# Autodesk Inventor assembly: gurav2 assembly
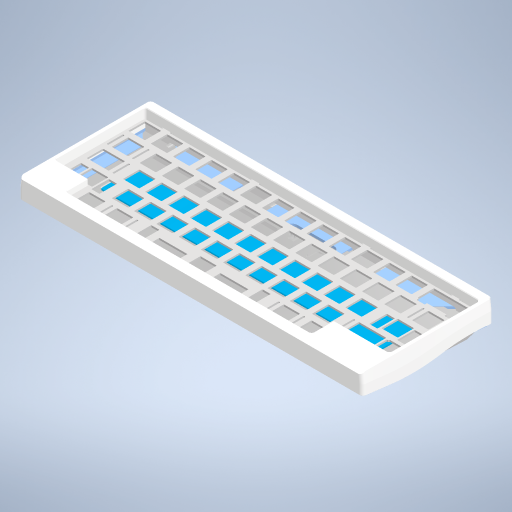
[picture p0: Inventor's stored thumbnail of the model, 512x512]
Saved by Autodesk Inventor 2023 (Build 270158000, 158)
## iProperties
Created: 2023-10-18
Part Number: gurav2 assembly
Document SubType Name: Assembly
Designer: Eric
Author: Eric
## Documents named in this file (8)
- C:\Users\Eric\Desktop\guracase\v2 Parts\gurav2 assembly.iam
- C:\Users\Eric\Desktop\guracase\v2 Parts\bottomcase.ipt
- C:\Users\Eric\Desktop\guracase\v2 Parts\rightdiffuser.ipt
- C:\Users\Eric\Desktop\guracase\v2 Parts\leftdiffuser.ipt
- C:\Users\Eric\Desktop\guracase\v2 Parts\reardiffuser.ipt
- C:\Users\Eric\Desktop\guracase\v2 Parts\weight.ipt
- C:\Users\Eric\Desktop\guracase\v2 Parts\topcase.ipt
- C:\Users\Eric\Desktop\guracase\v2 Parts\hhkbplate.ipt
## Components (7 placed, 7 different names)
1. bottomcase:1 — Mate:1, Mate:2, Mate:3, Mate:4, Mate:5, Mate:6, Mate:7, Mate:8, Flush:1, Mate:9, Mate:10, Flush:2, Mate:11, Mate:13
2. rightdiffuser:1 — Mate:1, Mate:2, Mate:3, Mate:12
3. leftdiffuser:1 — Mate:4, Mate:5, Mate:6
4. reardiffuser:1 — Mate:7, Mate:8, Flush:1
5. weight:1 — Mate:9, Mate:10, Flush:2
6. topcase:1 — Mate:11, Mate:12, Mate:13, Mate:14, Mate:15
7. hhkbplate:1 — Mate:14, Mate:15
## Relationships (17: Mate 15, Flush 2)
- Mate:1: bottomcase:1 ↔ rightdiffuser:1
- Mate:2 (0.125 mm): bottomcase:1 ↔ rightdiffuser:1
- Mate:3 (0.125 mm): bottomcase:1 ↔ rightdiffuser:1
- Mate:4: bottomcase:1 ↔ leftdiffuser:1
- Mate:5 (0.125 mm): bottomcase:1 ↔ leftdiffuser:1
- Mate:6 (0.125 mm): bottomcase:1 ↔ leftdiffuser:1
- Mate:7: bottomcase:1 ↔ reardiffuser:1
- Mate:8 (0.125 mm): bottomcase:1 ↔ reardiffuser:1
- Flush:1: bottomcase:1 ↔ reardiffuser:1
- Mate:9 (0.125 mm): bottomcase:1 ↔ weight:1
- Mate:10 (0.125 mm): bottomcase:1 ↔ weight:1
- Flush:2: bottomcase:1 ↔ weight:1
- Mate:11: bottomcase:1 ↔ topcase:1
- Mate:12 (0.125 mm): rightdiffuser:1 ↔ topcase:1
- Mate:13 (0.125 mm): bottomcase:1 ↔ topcase:1
- Mate:14: topcase:1 ↔ hhkbplate:1
- Mate:15: topcase:1 ↔ hhkbplate:1
